# Autodesk Inventor assembly: 000100
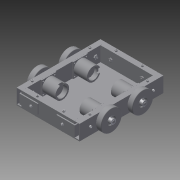
[picture p0: Inventor's stored thumbnail of the model, 180x180]
Saved by Autodesk Inventor 2015 (Build 190159000, 159)
## iProperties
Created: 2015-05-18
Part Number: 000100
Document SubType Name: Assembly
Designer: Wesley
Author: Wesley
## Documents named in this file (13)
- C:\Users\Wesley\Documents\GitHub\EngineeringFinal\Engineering\Engineering Documentation\CADS\0001__\000100.iam
- C:\Users\Wesley\Documents\GitHub\EngineeringFinal\Engineering\Engineering Documentation\CADS\0001__\000101-1.ipt
- C:\Users\Wesley\Documents\GitHub\EngineeringFinal\Engineering\Engineering Documentation\CADS\0001__\000101-2.ipt
- C:\Users\Wesley\Documents\GitHub\EngineeringFinal\Engineering\Engineering Documentation\CADS\0001__\000102.ipt
- C:\Users\Wesley\Documents\GitHub\EngineeringFinal\Engineering\Engineering Documentation\CADS\0001__\000103.ipt
- C:\Users\Wesley\Documents\GitHub\EngineeringFinal\Engineering\Engineering Documentation\CADS\0001__\000104.ipt
- C:\Users\Wesley\Documents\GitHub\EngineeringFinal\Engineering\Engineering Documentation\CADS\0001__\000108.ipt
- C:\Users\Wesley\Documents\GitHub\EngineeringFinal\Engineering\Engineering Documentation\CADS\0001__\000109.ipt
- C:\Users\Wesley\Documents\GitHub\EngineeringFinal\Engineering\Engineering Documentation\CADS\0001__\000107-1.ipt
- C:\Users\Wesley\Documents\GitHub\EngineeringFinal\Engineering\Engineering Documentation\CADS\0001__\000110.ipt
- C:\Users\Wesley\Documents\GitHub\EngineeringFinal\Engineering\Engineering Documentation\CADS\0001__\000106.ipt
- C:\Users\Wesley\Documents\GitHub\EngineeringFinal\Engineering\Engineering Documentation\CADS\0001__\000105-2.ipt
- C:\Users\Wesley\Documents\GitHub\EngineeringFinal\Engineering\Engineering Documentation\CADS\0001__\000105-1.ipt
## Components (61 placed, 12 different names)
1. 000101-1:1 — Mate:1, Flush:1, Flush:2, Flush:6, Mate:3, Mate:5, Mate:10, Mate:12, Mate:16, Flush:9, Mate:17, Mate:23, Mate:34, Mate:36, Mate:38, Mate:40, Mate:105, Mate:106, Mate:107, Mate:108, Mate:122, Mate:123, Mate:124, Mate:125, Mate:127, Mate:131
2. 000101-2:1 — Mate:1, Flush:1, Flush:2, Mate:2, Flush:3, Flush:4, Mate:4, Mate:6, Mate:7, Mate:11, Mate:69, Mate:70, Mate:76, Mate:77, Mate:78, Mate:98
3. 000101-1:2 — Mate:2, Flush:3, Flush:4, Flush:7, Mate:8, Mate:14, Mate:18, Mate:47, Mate:48, Mate:52, Mate:53, Mate:58, Mate:60, Mate:101, Mate:102, Mate:103, Mate:104, Mate:116, Mate:118, Mate:119, Mate:120, Mate:121, Mate:129, Mate:133
4. 000101-2:2 — Flush:6, Mate:3, Flush:7, Mate:9, Mate:13, Mate:15, Flush:8, Mate:79, Mate:80, Mate:81, Mate:82, Mate:91, Mate:92, Mate:99, Mate:100
5. 000102:1 — Mate:4, Mate:5, Mate:6, Mate:73, Mate:74
6. 000102:2 — Mate:9, Mate:10, Mate:12, Mate:94
7. 000102:3 — Mate:7, Mate:8, Mate:11, Mate:89, Mate:90
8. 000102:4 — Mate:13, Mate:14, Mate:15, Mate:93
9. 000103:1 — Mate:16, Flush:8, Flush:9, Mate:17, Mate:18, Mate:35, Mate:37, Mate:49, Mate:54, Mate:68, Mate:71, Mate:84, Mate:86, Mate:87, Mate:110, Mate:112, Mate:115, Mate:117
10. 000104:1 — Mate:59, Mate:60, Mate:61
11. 000104:2 — Mate:39, Mate:40, Mate:41, Mate:42
12. 000104:3 — Mate:19, Mate:26, Mate:27
13. 000104:4 — Mate:57, Mate:58, Mate:63
14. 000108:1 — Mate:19, Mate:21, Mate:22
15. 000109:1 — Mate:21, Mate:22, Mate:23, Mate:32, Mate:33
16. 000107-1:1 — Mate:26, Mate:27
17. 000109:2 — Mate:43, Mate:44, Mate:46
18. 000109:3 — Mate:28, Mate:29, Mate:30, Mate:31
19. 000109:4 — Mate:50, Mate:51, Mate:56
20. 000108:2 — Mate:55, Mate:56
21. 000108:3 — Mate:45, Mate:46
22. 000108:4 — Mate:28, Mate:29
23. 000110:1 — Mate:30, Mate:31, Mate:36, Mate:37, Mate:38, Mate:39
24. 000110:2 — Mate:32, Mate:33, Mate:34, Mate:35
25. 000107-1:2 — Mate:41, Mate:42
26. 000110:3 — Mate:43, Mate:44, Mate:45, Mate:47, Mate:48, Mate:49, Mate:59, Mate:62
27. 000110:4 — Mate:50, Mate:51, Mate:52, Mate:53, Mate:54, Mate:55, Mate:57, Mate:64
28. 000107-1:3 — Mate:61, Mate:62
29. 000107-1:4 — Mate:63, Mate:64
30. 000106:1 — Mate:68, Mate:71, Mate:72
31. 000105-2:1 — Mate:69, Mate:70, Mate:72
32. 000105-1:1 — Mate:73, Mate:74, Mate:75
33. 000106:2 — Mate:75, Mate:76
34. 000105-2:2 — Mate:77, Mate:78, Mate:83
35. 000105-2:3 — Mate:80, Mate:81, Mate:85
36. 000105-2:4 — Mate:79, Mate:82, Mate:88
37. 000106:3 — Mate:83, Mate:84
38. 000106:4 — Mate:85, Mate:86
39. 000106:5 — Mate:87, Mate:88
40. 000105-1:2 — Mate:89, Mate:90, Mate:97
41. 000105-1:3 — Mate:92, Mate:93, Mate:95
42. 000105-1:4 — Mate:91, Mate:94, Mate:96
43. 000106:6 — Mate:97, Mate:98
44. 000106:7 — Mate:96, Mate:100
45. 000106:8 — Mate:95, Mate:99
46. 000105-2:5 — Mate:101, Mate:102
47. 000105-2:6 — Mate:106, Mate:108, Mate:111
48. 000105-2:7 — Mate:105, Mate:107, Mate:109
49. 000105-2:8 — Mate:103, Mate:104, Mate:114
50. 000106:9 — Mate:114, Mate:115
51. 000106:11 — Mate:109, Mate:110
52. 000106:12 — Mate:111, Mate:112
53. 000106:13 — Mate:116, Mate:117
54. 000105-1:5 — Mate:124, Mate:125, Mate:126
55. 000105-1:6 — Mate:120, Mate:121, Mate:132
56. 000105-1:7 — Mate:118, Mate:119, Mate:128
57. 000105-1:8 — Mate:122, Mate:123, Mate:130
58. 000106:14 — Mate:126, Mate:127
59. 000106:15 — Mate:130, Mate:131
60. 000106:16 — Mate:132, Mate:133
61. 000106:17 — Mate:128, Mate:129
## Relationships (134: Mate 126, Flush 8)
- Mate:1: 000101-1:1 ↔ 000101-2:1
- Flush:1: 000101-1:1 ↔ 000101-2:1
- Flush:2: 000101-1:1 ↔ 000101-2:1
- Mate:2: 000101-2:1 ↔ 000101-1:2
- Flush:3: 000101-2:1 ↔ 000101-1:2
- Flush:4: 000101-2:1 ↔ 000101-1:2
- Flush:6: 000101-1:1 ↔ 000101-2:2
- Mate:3: 000101-1:1 ↔ 000101-2:2
- Flush:7: 000101-1:2 ↔ 000101-2:2
- Mate:4: 000101-2:1 ↔ 000102:1
- Mate:5: 000101-1:1 ↔ 000102:1
- Mate:6: 000101-2:1 ↔ 000102:1
- Mate:7: 000101-2:1 ↔ 000102:3
- Mate:8: 000101-1:2 ↔ 000102:3
- Mate:9: 000101-2:2 ↔ 000102:2
- Mate:10: 000101-1:1 ↔ 000102:2
- Mate:11: 000101-2:1 ↔ 000102:3
- Mate:12: 000101-1:1 ↔ 000102:2
- Mate:13: 000101-2:2 ↔ 000102:4
- Mate:14: 000101-1:2 ↔ 000102:4
- Mate:15: 000101-2:2 ↔ 000102:4
- Mate:16: 000101-1:1 ↔ 000103:1
- Flush:8: 000101-2:2 ↔ 000103:1
- Flush:9: 000101-1:1 ↔ 000103:1
- Mate:17: 000101-1:1 ↔ 000103:1
- Mate:18: 000101-1:2 ↔ 000103:1
- Mate:19: 000104:3 ↔ 000108:1
- Mate:21: 000108:1 ↔ 000109:1
- Mate:22: 000108:1 ↔ 000109:1
- Mate:23: 000101-1:1 ↔ 000109:1
- Mate:26: 000104:3 ↔ 000107-1:1
- Mate:27: 000104:3 ↔ 000107-1:1
- Mate:28: 000109:3 ↔ 000108:4
- Mate:29: 000109:3 ↔ 000108:4
- Mate:30: 000109:3 ↔ 000110:1
- Mate:31: 000109:3 ↔ 000110:1
- Mate:32: 000109:1 ↔ 000110:2
- Mate:33: 000109:1 ↔ 000110:2
- Mate:34: 000101-1:1 ↔ 000110:2
- Mate:35: 000103:1 ↔ 000110:2
- Mate:36: 000101-1:1 ↔ 000110:1
- Mate:37: 000103:1 ↔ 000110:1
- Mate:38: 000101-1:1 ↔ 000110:1
- Mate:39: 000104:2 ↔ 000110:1
- Mate:40 (1.27 mm): 000101-1:1 ↔ 000104:2
- Mate:41: 000104:2 ↔ 000107-1:2
- Mate:42: 000104:2 ↔ 000107-1:2
- Mate:43: 000109:2 ↔ 000110:3
- Mate:44: 000109:2 ↔ 000110:3
- Mate:45: 000108:3 ↔ 000110:3
- Mate:46: 000109:2 ↔ 000108:3
- Mate:47: 000101-1:2 ↔ 000110:3
- Mate:48: 000101-1:2 ↔ 000110:3
- Mate:49: 000103:1 ↔ 000110:3
- Mate:50: 000109:4 ↔ 000110:4
- Mate:51: 000109:4 ↔ 000110:4
- Mate:52: 000101-1:2 ↔ 000110:4
- Mate:53: 000101-1:2 ↔ 000110:4
- Mate:54: 000103:1 ↔ 000110:4
- Mate:55: 000108:2 ↔ 000110:4
- Mate:56: 000109:4 ↔ 000108:2
- Mate:57: 000104:4 ↔ 000110:4
- Mate:58 (1.27 mm): 000101-1:2 ↔ 000104:4
- Mate:59: 000104:1 ↔ 000110:3
- Mate:60 (1.27 mm): 000101-1:2 ↔ 000104:1
- Mate:61: 000104:1 ↔ 000107-1:3
- Mate:62: 000110:3 ↔ 000107-1:3
- Mate:63: 000104:4 ↔ 000107-1:4
- Mate:64: 000110:4 ↔ 000107-1:4
- Mate:68: 000103:1 ↔ 000106:1
- Mate:69: 000101-2:1 ↔ 000105-2:1
- Mate:70: 000101-2:1 ↔ 000105-2:1
- Mate:71: 000103:1 ↔ 000106:1
- Mate:72: 000106:1 ↔ 000105-2:1
- Mate:73: 000102:1 ↔ 000105-1:1
- Mate:74: 000102:1 ↔ 000105-1:1
- Mate:75: 000105-1:1 ↔ 000106:2
- Mate:76: 000101-2:1 ↔ 000106:2
- Mate:77: 000101-2:1 ↔ 000105-2:2
- Mate:78: 000101-2:1 ↔ 000105-2:2
- Mate:79: 000101-2:2 ↔ 000105-2:4
- Mate:80: 000101-2:2 ↔ 000105-2:3
- Mate:81: 000101-2:2 ↔ 000105-2:3
- Mate:82: 000101-2:2 ↔ 000105-2:4
- Mate:83: 000105-2:2 ↔ 000106:3
- Mate:84: 000103:1 ↔ 000106:3
- Mate:85: 000105-2:3 ↔ 000106:4
- Mate:86: 000103:1 ↔ 000106:4
- Mate:87: 000103:1 ↔ 000106:5
- Mate:88: 000105-2:4 ↔ 000106:5
- Mate:89: 000102:3 ↔ 000105-1:2
- Mate:90: 000102:3 ↔ 000105-1:2
- Mate:91: 000101-2:2 ↔ 000105-1:4
- Mate:92: 000101-2:2 ↔ 000105-1:3
- Mate:93: 000102:4 ↔ 000105-1:3
- Mate:94: 000102:2 ↔ 000105-1:4
- Mate:95: 000105-1:3 ↔ 000106:8
- Mate:96: 000105-1:4 ↔ 000106:7
- Mate:97: 000105-1:2 ↔ 000106:6
- Mate:98: 000101-2:1 ↔ 000106:6
- Mate:99: 000101-2:2 ↔ 000106:8
- Mate:100: 000101-2:2 ↔ 000106:7
- Mate:101: 000101-1:2 ↔ 000105-2:5
- Mate:102: 000101-1:2 ↔ 000105-2:5
- Mate:103: 000101-1:2 ↔ 000105-2:8
- Mate:104: 000101-1:2 ↔ 000105-2:8
- Mate:105: 000101-1:1 ↔ 000105-2:7
- Mate:106: 000101-1:1 ↔ 000105-2:6
- Mate:107: 000101-1:1 ↔ 000105-2:7
- Mate:108: 000101-1:1 ↔ 000105-2:6
- Mate:109: 000105-2:7 ↔ 000106:11
- Mate:110: 000103:1 ↔ 000106:11
- Mate:111: 000105-2:6 ↔ 000106:12
- Mate:112: 000103:1 ↔ 000106:12
- Mate:114: 000105-2:8 ↔ 000106:9
- Mate:115: 000103:1 ↔ 000106:9
- Mate:116: 000101-1:2 ↔ 000106:13
- Mate:117: 000103:1 ↔ 000106:13
- Mate:118: 000101-1:2 ↔ 000105-1:7
- Mate:119: 000101-1:2 ↔ 000105-1:7
- Mate:120: 000101-1:2 ↔ 000105-1:6
- Mate:121: 000101-1:2 ↔ 000105-1:6
- Mate:122: 000101-1:1 ↔ 000105-1:8
- Mate:123: 000101-1:1 ↔ 000105-1:8
- Mate:124: 000101-1:1 ↔ 000105-1:5
- Mate:125: 000101-1:1 ↔ 000105-1:5
- Mate:126: 000105-1:5 ↔ 000106:14
- Mate:127: 000101-1:1 ↔ 000106:14
- Mate:128: 000105-1:7 ↔ 000106:17
- Mate:129: 000101-1:2 ↔ 000106:17
- Mate:130: 000105-1:8 ↔ 000106:15
- Mate:131: 000101-1:1 ↔ 000106:15
- Mate:132: 000105-1:6 ↔ 000106:16
- Mate:133: 000101-1:2 ↔ 000106:16
